# Autodesk Inventor assembly: Monitor with Plugs
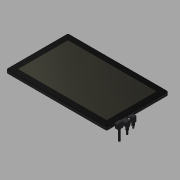
[picture p0: Inventor's stored thumbnail of the model, 180x180]
Saved by Autodesk Inventor 2019 (Build 230136000, 136)
## iProperties
Created: 2019-02-12
Part Number: Monitor with Plugs
Document SubType Name: Assembly
Designer: Ben
Author: Ben
## Documents named in this file (5)
- C:\Users\Ben\Documents\Inventor\HydraVivarium\Monitor with Plugs.iam
- C:\Users\Ben\Documents\Inventor\HydraVivarium\MageDok Screen.ipt
- C:\Users\Ben\Documents\Inventor\HydraVivarium\USB C Right Angle Plug.ipt
- C:\Users\Ben\Documents\Inventor\HydraVivarium\HDMI Mini Right Angle Plug.ipt
- C:\Users\Ben\Documents\Inventor\HydraVivarium\USB Micro Right Angle Plug.ipt
## Components (4 placed, 4 different names)
1. MageDok Screen:1 — Mate:1, Mate:2, Mate:3, Angle:1, Angle:2, Angle:3, Mate:4, Mate:5, Mate:6
2. USB C Right Angle Plug:1 — Mate:1, Angle:1, Mate:6
3. HDMI Mini Right Angle Plug:1 — Mate:2, Angle:2, Mate:5
4. USB Micro Right Angle Plug:1 — Mate:3, Angle:3, Mate:4
## Relationships (9: Mate 6, Angle 3)
- Mate:1: MageDok Screen:1 ↔ USB C Right Angle Plug:1
- Mate:2: MageDok Screen:1 ↔ HDMI Mini Right Angle Plug:1
- Mate:3: MageDok Screen:1 ↔ USB Micro Right Angle Plug:1
- Angle:1 (0 deg): MageDok Screen:1 ↔ USB C Right Angle Plug:1
- Angle:2 (0 deg): MageDok Screen:1 ↔ HDMI Mini Right Angle Plug:1
- Angle:3 (0 deg): MageDok Screen:1 ↔ USB Micro Right Angle Plug:1
- Mate:4 (2 mm): MageDok Screen:1 ↔ USB Micro Right Angle Plug:1
- Mate:5 (1.5 mm): MageDok Screen:1 ↔ HDMI Mini Right Angle Plug:1
- Mate:6 (2 mm): MageDok Screen:1 ↔ USB C Right Angle Plug:1
